# Autodesk Inventor assembly: assy_mission_parking_lot
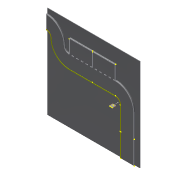
[picture p0: Inventor's stored thumbnail of the model, 180x180]
Saved by Autodesk Inventor 2018 (Build 220112000, 112)
## iProperties
Created: 2017-11-13
Part Number: assy_mission_parking_lot
Document SubType Name: Assembly
Designer: Platform
Author: Platform
## Documents named in this file (10)
- C:\Users\Platform\Desktop\autorace_track\track_model\autorace_rbizchallenge2017\assembled\assy_mission_parking_lot.iam
- C:\Users\Platform\Desktop\autorace_track\track_model\autorace_rbizchallenge2017\assembled\assy_lower_plates.iam
- C:\Users\Platform\Desktop\autorace_track\track_model\autorace_rbizchallenge2017\assembled\assy_straight.iam
- C:\Users\Platform\Desktop\autorace_track\track_model\autorace_rbizchallenge2017\assembled\assy_curved_left.iam
- C:\Users\Platform\Desktop\autorace_track\track_model\autorace_rbizchallenge2017\assembled\assy_parkinglot_front_left.iam
- C:\Users\Platform\Desktop\autorace_track\track_model\autorace_rbizchallenge2017\assembled\assy_parkinglot_rear_left.iam
- C:\Users\Platform\Desktop\autorace_track\track_model\autorace_rbizchallenge2017\assembled\assy_parkinglot_front_right.iam
- C:\Users\Platform\Desktop\autorace_track\track_model\autorace_rbizchallenge2017\assembled\assy_parkinglot_rear_right.iam
- C:\Users\Platform\Desktop\autorace_track\track_model\autorace_rbizchallenge2017\assembled\assy_curved_right.iam
- C:\Users\Platform\Desktop\autorace_track\track_model\autorace_rbizchallenge2017\parts\ipt\parking_sign.ipt
## Components (11 placed, 9 different names)
1. assy_lower_plates:1 [sub-assembly] — Mate:1, Flush:1, Flush:2, Mate:2, Mate:4, Mate:7, Mate:10, Mate:12, Mate:14, Mate:16, Mate:19, Mate:22, Mate:24
2. assy_straight:1 [sub-assembly] — Mate:1, Flush:1, Flush:2, Flush:3, Mate:3
3. assy_straight:2 [sub-assembly] — Mate:2, Flush:3, Mate:3, Mate:5, Mate:6, Mate:23
4. assy_curved_left:1 [sub-assembly] — Mate:4, Mate:5, Mate:6, Mate:8, Mate:9
5. assy_parkinglot_front_left:1 [sub-assembly] — Mate:7, Mate:8, Mate:9, Mate:11, Flush:4, Mate:13, Flush:5
6. assy_parkinglot_rear_left:1 [sub-assembly] — Mate:10, Mate:11, Flush:4, Mate:15, Flush:6, Mate:17, Mate:18
7. assy_parkinglot_front_right:1 [sub-assembly] — Mate:12, Mate:13, Flush:5
8. assy_parkinglot_rear_right:1 [sub-assembly] — Mate:14, Mate:15, Flush:6
9. assy_curved_right:1 [sub-assembly] — Mate:16, Mate:17, Mate:18, Mate:20, Mate:21
10. assy_curved_left:2 [sub-assembly] — Mate:19, Mate:20, Mate:21
11. parking_sign:1 — Mate:22, Mate:23, Mate:24
## Relationships (30: Mate 24, Flush 6)
- Mate:1: assy_lower_plates:1 ↔ assy_straight:1
- Flush:1: assy_lower_plates:1 ↔ assy_straight:1
- Flush:2 (100 mm): assy_lower_plates:1 ↔ assy_straight:1
- Mate:2: assy_lower_plates:1 ↔ assy_straight:2
- Flush:3: assy_straight:1 ↔ assy_straight:2
- Mate:3: assy_straight:1 ↔ assy_straight:2
- Mate:4: assy_lower_plates:1 ↔ assy_curved_left:1
- Mate:5: assy_straight:2 ↔ assy_curved_left:1
- Mate:6: assy_straight:2 ↔ assy_curved_left:1
- Mate:7: assy_lower_plates:1 ↔ assy_parkinglot_front_left:1
- Mate:8: assy_curved_left:1 ↔ assy_parkinglot_front_left:1
- Mate:9: assy_curved_left:1 ↔ assy_parkinglot_front_left:1
- Mate:10: assy_lower_plates:1 ↔ assy_parkinglot_rear_left:1
- Mate:11: assy_parkinglot_front_left:1 ↔ assy_parkinglot_rear_left:1
- Flush:4: assy_parkinglot_front_left:1 ↔ assy_parkinglot_rear_left:1
- Mate:12: assy_lower_plates:1 ↔ assy_parkinglot_front_right:1
- Mate:13: assy_parkinglot_front_left:1 ↔ assy_parkinglot_front_right:1
- Flush:5: assy_parkinglot_front_left:1 ↔ assy_parkinglot_front_right:1
- Mate:14: assy_lower_plates:1 ↔ assy_parkinglot_rear_right:1
- Mate:15: assy_parkinglot_rear_left:1 ↔ assy_parkinglot_rear_right:1
- Flush:6: assy_parkinglot_rear_left:1 ↔ assy_parkinglot_rear_right:1
- Mate:16: assy_lower_plates:1 ↔ assy_curved_right:1
- Mate:17: assy_parkinglot_rear_left:1 ↔ assy_curved_right:1
- Mate:18: assy_parkinglot_rear_left:1 ↔ assy_curved_right:1
- Mate:19: assy_lower_plates:1 ↔ assy_curved_left:2
- Mate:20: assy_curved_right:1 ↔ assy_curved_left:2
- Mate:21: assy_curved_right:1 ↔ assy_curved_left:2
- Mate:22: assy_lower_plates:1 ↔ parking_sign:1
- Mate:23 (50 mm): assy_straight:2 ↔ parking_sign:1
- Mate:24: assy_lower_plates:1 ↔ parking_sign:1
